# Autodesk Inventor assembly: DroneAssembly
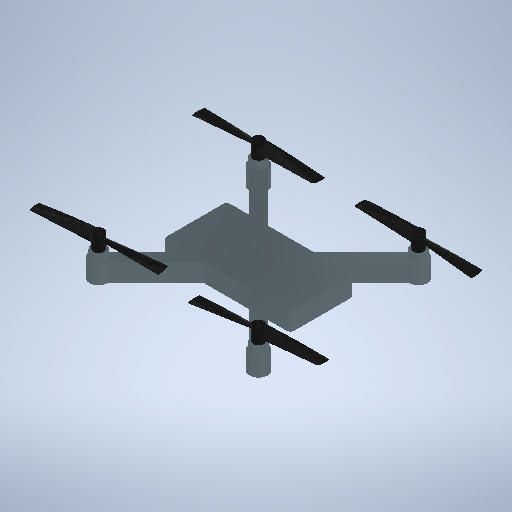
[picture p0: Inventor's stored thumbnail of the model, 512x512]
Saved by Autodesk Inventor 2025.1 (Build 291241000, 241)
## iProperties
Created: 2024-10-02
Part Number: DroneAssembly
Document SubType Name: Assembly
Designer: fears
Author: fears
## Documents named in this file (4)
- D:\Documents\University\Year4\DroneProject\DroneGroupProject\3DModels\Inventor\DroneAssembly.iam
- D:\Documents\University\Year4\DroneProject\DroneGroupProject\3DModels\Inventor\DroneBase.ipt
- D:\Documents\University\Year4\DroneProject\DroneGroupProject\3DModels\Inventor\BladeCW.ipt
- D:\Documents\University\Year4\DroneProject\DroneGroupProject\3DModels\Inventor\BladeCCW.ipt
## Components (5 placed, 3 different names)
1. DroneBase:1 — Rotational:1, Rotational:2, Rotational:3, Rotational:4
2. BladeCW:1 — Rotational:1
3. BladeCW:2 — Rotational:2
4. BladeCCW:1 — Rotational:4
5. BladeCCW:2 — Rotational:3
## Relationships (4: RevoluteJoint 4)
- Rotational:1 [RevoluteJoint]: DroneBase:1 ↔ BladeCW:1
- Rotational:2 [RevoluteJoint]: DroneBase:1 ↔ BladeCW:2
- Rotational:3 [RevoluteJoint]: DroneBase:1 ↔ BladeCCW:2
- Rotational:4 [RevoluteJoint]: DroneBase:1 ↔ BladeCCW:1
